# Autodesk Inventor assembly: F_Foot
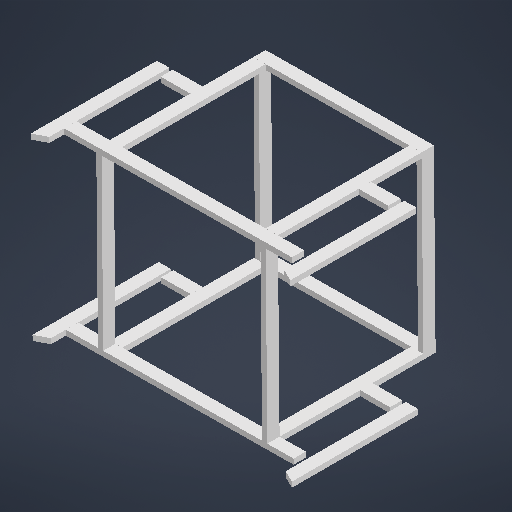
[picture p0: Inventor's stored thumbnail of the model, 512x512]
Saved by Autodesk Inventor 2026 (Build 300175000, 175)
## iProperties
Created: 2025-09-08
Part Number: F_Foot
Document SubType Name: Assembly
Designer: trott
Author: trott
## Documents named in this file (6)
- C:\Users\trott\Documents\UofSC-ASME-Tiger-Burn-Design-2025\CAD\Legs\Front Foot\F_Foot.iam
- C:\Users\trott\Documents\UofSC-ASME-Tiger-Burn-Design-2025\CAD\Legs\Front Foot\2x4x48.ipt
- C:\Users\trott\Documents\UofSC-ASME-Tiger-Burn-Design-2025\CAD\Legs\Front Foot\2x4x41.ipt
- C:\Users\trott\Documents\UofSC-ASME-Tiger-Burn-Design-2025\CAD\Legs\Front Foot\2x4x67.ipt
- C:\Users\trott\Documents\UofSC-ASME-Tiger-Burn-Design-2025\CAD\Legs\Front Foot\2x4x8.5.ipt
- C:\Users\trott\Documents\UofSC-ASME-Tiger-Burn-Design-2025\CAD\Legs\Front Foot\S_2x4x36.ipt
## Components (20 placed, 5 different names)
1. 2x4x48:1 — Mate:1, Mate:2, Mate:3, Mate:4, Mate:7, Mate:8, Mate:11
2. 2x4x48:2 — Mate:1, Mate:2, Mate:5, Mate:6, Flush:15
3. 2x4x48:3 — Mate:3, Mate:4
4. 2x4x48:4 — Mate:5, Mate:6, Mate:19, Mate:20, Mate:21, Mate:27, Mate:28, Flush:19, Flush:20
5. 2x4x41:1 — Mate:7, Mate:8, Mate:26, Flush:5
6. 2x4x41:2 — Mate:11, Mate:30, Flush:9, Flush:11, Flush:13
7. 2x4x41:3 — Mate:19, Mate:20, Mate:22, Flush:1, Flush:2, Mate:24, Flush:4, Flush:20, Flush:21
8. 2x4x41:4 — Mate:21, Mate:27, Mate:28, Mate:29, Flush:7, Flush:18, Flush:19
9. 2x4x67:1 — Mate:22, Flush:1, Flush:2, Flush:3, Mate:25, Mate:31, Mate:33, Mate:34, Flush:18, Flush:21
10. 2x4x67:2 — Flush:3, Flush:11, Mate:36, Flush:12, Mate:37, Flush:14, Mate:38, Mate:39, Flush:22
11. 2x4x8.5:1 — Mate:24, Flush:4, Mate:25, Flush:6, Flush:8, Mate:32
12. 2x4x8.5:2 — Mate:26, Flush:5, Flush:6, Flush:10, Flush:23
13. 2x4x8.5:3 — Mate:29, Flush:7, Flush:8, Mate:35
14. 2x4x8.5:4 — Mate:30, Flush:9, Flush:10, Flush:16, Flush:17
15. S_2x4x36:1 — Mate:31, Mate:32
16. S_2x4x36:2 — Mate:33, Mate:34, Mate:35
17. 2x4x48:5 — Mate:36, Flush:12, Flush:13
18. 2x4x48:6 — Mate:37, Flush:14, Flush:15
19. S_2x4x36:3 — Mate:38, Flush:16, Flush:17
20. S_2x4x36:4 — Mate:39, Flush:22, Flush:23
## Relationships (52: Mate 29, Flush 23)
- Mate:1: 2x4x48:1 ↔ 2x4x48:2
- Mate:2: 2x4x48:1 ↔ 2x4x48:2
- Mate:3: 2x4x48:1 ↔ 2x4x48:3
- Mate:4: 2x4x48:1 ↔ 2x4x48:3
- Mate:5: 2x4x48:2 ↔ 2x4x48:4
- Mate:6: 2x4x48:2 ↔ 2x4x48:4
- Mate:7: 2x4x48:1 ↔ 2x4x41:1
- Mate:8: 2x4x48:1 ↔ 2x4x41:1
- Mate:11: 2x4x48:1 ↔ 2x4x41:2
- Mate:19: 2x4x48:4 ↔ 2x4x41:3
- Mate:20: 2x4x48:4 ↔ 2x4x41:3
- Mate:21: 2x4x48:4 ↔ 2x4x41:4
- Mate:22: 2x4x41:3 ↔ 2x4x67:1
- Flush:1 (-241.3 mm): 2x4x41:3 ↔ 2x4x67:1
- Flush:2: 2x4x41:3 ↔ 2x4x67:1
- Flush:3: 2x4x67:1 ↔ 2x4x67:2
- Mate:24: 2x4x41:3 ↔ 2x4x8.5:1
- Flush:4: 2x4x41:3 ↔ 2x4x8.5:1
- Mate:25 (-762 mm): 2x4x67:1 ↔ 2x4x8.5:1
- Mate:26: 2x4x41:1 ↔ 2x4x8.5:2
- Flush:5: 2x4x41:1 ↔ 2x4x8.5:2
- Flush:6: 2x4x8.5:1 ↔ 2x4x8.5:2
- Mate:27: 2x4x48:4 ↔ 2x4x41:4
- Mate:28: 2x4x48:4 ↔ 2x4x41:4
- Mate:29: 2x4x41:4 ↔ 2x4x8.5:3
- Flush:7: 2x4x41:4 ↔ 2x4x8.5:3
- Flush:8: 2x4x8.5:1 ↔ 2x4x8.5:3
- Mate:30: 2x4x41:2 ↔ 2x4x8.5:4
- Flush:9: 2x4x41:2 ↔ 2x4x8.5:4
- Flush:10: 2x4x8.5:2 ↔ 2x4x8.5:4
- Mate:31: 2x4x67:1 ↔ S_2x4x36:1
- Mate:32: 2x4x8.5:1 ↔ S_2x4x36:1
- Mate:33: 2x4x67:1 ↔ S_2x4x36:2
- Mate:34: 2x4x67:1 ↔ S_2x4x36:2
- Mate:35: 2x4x8.5:3 ↔ S_2x4x36:2
- Flush:11: 2x4x41:2 ↔ 2x4x67:2
- Mate:36: 2x4x67:2 ↔ 2x4x48:5
- Flush:12: 2x4x67:2 ↔ 2x4x48:5
- Flush:13: 2x4x41:2 ↔ 2x4x48:5
- Mate:37: 2x4x67:2 ↔ 2x4x48:6
- Flush:14: 2x4x67:2 ↔ 2x4x48:6
- Flush:15: 2x4x48:2 ↔ 2x4x48:6
- Mate:38: 2x4x67:2 ↔ S_2x4x36:3
- Flush:16: 2x4x8.5:4 ↔ S_2x4x36:3
- Flush:17: 2x4x8.5:4 ↔ S_2x4x36:3
- Flush:18: 2x4x41:4 ↔ 2x4x67:1
- Flush:19: 2x4x48:4 ↔ 2x4x41:4
- Flush:20: 2x4x48:4 ↔ 2x4x41:3
- Flush:21: 2x4x41:3 ↔ 2x4x67:1
- Mate:39: 2x4x67:2 ↔ S_2x4x36:4
- Flush:22: 2x4x67:2 ↔ S_2x4x36:4
- Flush:23: 2x4x8.5:2 ↔ S_2x4x36:4
